# Autodesk Inventor assembly: gimbal
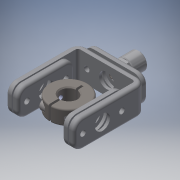
[picture p0: Inventor's stored thumbnail of the model, 180x180]
Saved by Autodesk Inventor 2019 (Build 230136000, 136)
## iProperties
Created: 2018-08-03
Part Number: gimbal
Document SubType Name: Assembly
Designer: Brian
Author: Brian
## Documents named in this file (6)
- C:\Users\Brian\Desktop\designs\gimbal\gimbal.iam
- C:\Users\Brian\Desktop\designs\gimbal\top.ipt
- C:\Users\Brian\Desktop\designs\gimbal\sides.ipt
- C:\Users\Brian\Desktop\designs\gimbal\bottom_v2.ipt
- C:\Users\Brian\Desktop\designs\gimbal\Ruland_OH-MCL-12-A\Ruland_OH-MCL-12-A.iam
- C:\Users\Brian\Desktop\designs\gimbal\TH060-Step.ipt
## Components (6 placed, 5 different names)
1. top:1 — Mate:2, Flush:2, Flush:3, Mate:3, Flush:4, Flush:5, Mate:4, Flush:6, Mate:5
2. sides:1 — Mate:2, Flush:2, Flush:3
3. sides:2 — Mate:3, Flush:4, Flush:5
4. bottom_v2:1 — Mate:4, Flush:6, Mate:5, Mate:6
5. Ruland_OH-MCL-12-A:1 [sub-assembly]
6. TH060-Step:1 — Mate:6
## Relationships (10: Mate 5, Flush 5)
- Mate:2 (1 mm): top:1 ↔ sides:1
- Flush:2: top:1 ↔ sides:1
- Flush:3: top:1 ↔ sides:1
- Mate:3 (1 mm): top:1 ↔ sides:2
- Flush:4: top:1 ↔ sides:2
- Flush:5: top:1 ↔ sides:2
- Mate:4 (1 mm): top:1 ↔ bottom_v2:1
- Flush:6: top:1 ↔ bottom_v2:1
- Mate:5: top:1 ↔ bottom_v2:1
- Mate:6: bottom_v2:1 ↔ TH060-Step:1
